# Autodesk Inventor assembly: Main Assembly
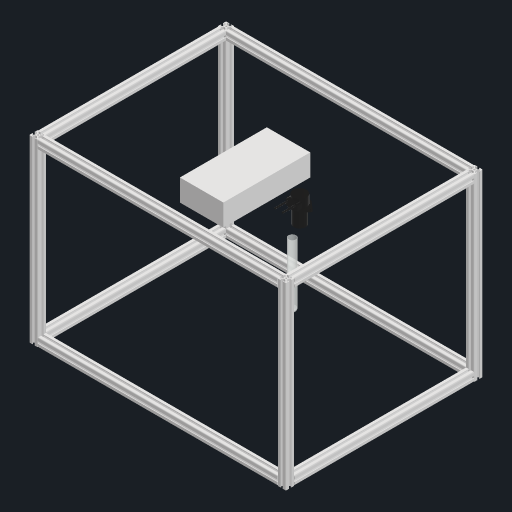
[picture p0: Inventor's stored thumbnail of the model, 512x512]
Saved by Autodesk Inventor 2023.1 (Build 271208000, 208)
## iProperties
Created: 2022-10-27
Part Number: Main Assembly
Document SubType Name: Assembly
Designer: JARRETT
Author: JARRETT
## Documents named in this file (6)
- C:\Users\Jarrett\Desktop\Projects\BehrendURCMechanical\CAD\Science\Main Assembly.iam
- C:\Users\Jarrett\Desktop\Projects\BehrendURCMechanical\CAD\Science\8020 Frame Horizontal.ipt
- C:\Users\Jarrett\Desktop\Projects\BehrendURCMechanical\CAD\Science\8020 Frame Vertical.ipt
- C:\Users\Jarrett\Desktop\Projects\BehrendURCMechanical\CAD\Science\Test Tube.ipt
- C:\Users\Jarrett\Desktop\Projects\BehrendURCMechanical\CAD\Science\Styrofoam.ipt
- C:\Users\Jarrett\Desktop\Projects\BehrendURCMechanical\CAD\Science\Peristaltic Pump.ipt
## Components (15 placed, 5 different names)
1. 8020 Frame Horizontal:1 — Rigid:1, Rigid:2
2. 8020 Frame Vertical:1 — Rigid:1, Rigid:9, Rigid:14, Rigid:15
3. 8020 Frame Vertical:2 — Rigid:2, Rigid:12, Rigid:13
4. 8020 Frame Vertical:3 — Rigid:5
5. 8020 Frame Vertical:4 — Rigid:6, Rigid:11, Rigid:16
6. 8020 Frame Horizontal:4 — Rigid:5, Rigid:6
7. 8020 Frame Horizontal:6 — Rigid:9
8. 8020 Frame Horizontal:8 — Rigid:11
9. Test Tube:1
10. Styrofoam:1
11. Peristaltic Pump:1
12. 8020 Frame Vertical:5 — Rigid:12
13. 8020 Frame Vertical:6 — Rigid:13
14. 8020 Frame Vertical:7 — Rigid:14
15. 8020 Frame Vertical:8 — Rigid:15, Rigid:16
## Relationships (11: WeldJoint 11)
- Rigid:1 [WeldJoint]: 8020 Frame Horizontal:1 ↔ 8020 Frame Vertical:1
- Rigid:2 [WeldJoint]: 8020 Frame Horizontal:1 ↔ 8020 Frame Vertical:2
- Rigid:5 [WeldJoint]: 8020 Frame Vertical:3 ↔ 8020 Frame Horizontal:4
- Rigid:6 [WeldJoint]: 8020 Frame Vertical:4 ↔ 8020 Frame Horizontal:4
- Rigid:9 [WeldJoint]: 8020 Frame Vertical:1 ↔ 8020 Frame Horizontal:6
- Rigid:11 [WeldJoint]: 8020 Frame Vertical:4 ↔ 8020 Frame Horizontal:8
- Rigid:12 [WeldJoint]: 8020 Frame Vertical:2 ↔ 8020 Frame Vertical:5
- Rigid:13 [WeldJoint]: 8020 Frame Vertical:2 ↔ 8020 Frame Vertical:6
- Rigid:14 [WeldJoint]: 8020 Frame Vertical:1 ↔ 8020 Frame Vertical:7
- Rigid:15 [WeldJoint]: 8020 Frame Vertical:1 ↔ 8020 Frame Vertical:8
- Rigid:16 [WeldJoint]: 8020 Frame Vertical:4 ↔ 8020 Frame Vertical:8
